# Autodesk Inventor assembly: ASY MSC 900.4  base frame
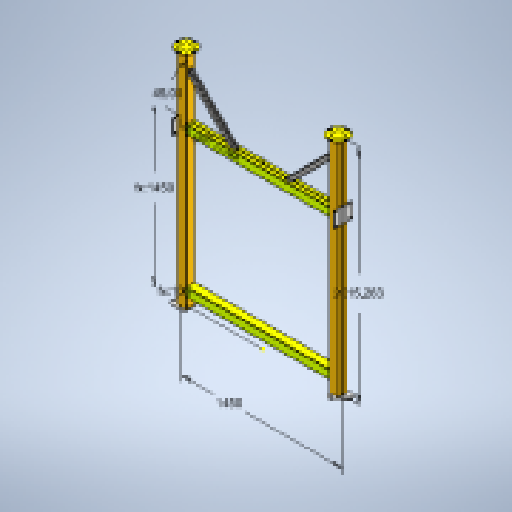
[picture p0: Inventor's stored thumbnail of the model, 512x512]
Saved by Autodesk Inventor 2025 (Build 290162010, 162A)
## iProperties
Created: 2024-06-30
Part Number: ASY MSC 900.4  base frame
Document SubType Name: Assembly
Designer: pokla
Stock Number: ASY МОО 900.4 базовая рама
_SolveAssemblyDoc: Frame Generator Solve Assembly
_Version: 25.0.0
Author: pokla
## Documents named in this file (7)
- C:\Users\pokla\Documents\Inventor\Отстойник осветлитель\Manturovo_Se-clar-Gleb\Pillars\ASY MSC 900.4  base frame.iam
- C:\Users\pokla\Documents\Inventor\Отстойник осветлитель\Manturovo_Se-clar-Gleb\Pillars\MSC DIM 009.4 base frame sketch.ipt
- C:\Users\pokla\Documents\Inventor\Отстойник осветлитель\Manturovo_Se-clar-Gleb\MSC 902 flange frame heel.ipt
- C:\Users\pokla\Documents\Inventor\Отстойник осветлитель\Manturovo_Se-clar-Gleb\MSC 906 flange frame.ipt
- C:\Users\pokla\Documents\Inventor\Отстойник осветлитель\Manturovo_Se-clar-Gleb\Pillars\Frame 1725454009874.iam
- C:\Users\pokla\Documents\Inventor\Отстойник осветлитель\Manturovo_Se-clar-Gleb\MSC DIM 000 settler-clarifier.ipt
- C:\Users\pokla\Documents\Inventor\Отстойник осветлитель\Manturovo_Se-clar-Gleb\MSC 908 transverse pillar plate.ipt
## Components (9 placed, 6 different names)
1. MSC DIM 009.4 base frame sketch:1
2. MSC 902 flange frame heel:1 — Rigid:2
3. MSC 902 flange frame heel:2 — Rigid:3
4. MSC 906 flange frame:1 — Rigid:4
5. MSC 906 flange frame:2 — Rigid:1
6. Frame 1725454009874:1 [sub-assembly] — Rigid:1, Rigid:2, Rigid:3, Rigid:4, Rigid:5, Rigid:6
7. MSC DIM 000 settler-clarifier:1
8. MSC 908 transverse pillar plate:1 — Rigid:5
9. MSC 908 transverse pillar plate:2 — Rigid:6
## Relationships (6: WeldJoint 6)
- Rigid:1 [WeldJoint]: MSC 906 flange frame:2 ↔ Frame 1725454009874:1
- Rigid:2 [WeldJoint]: MSC 902 flange frame heel:1 ↔ Frame 1725454009874:1
- Rigid:3 [WeldJoint]: MSC 902 flange frame heel:2 ↔ Frame 1725454009874:1
- Rigid:4 [WeldJoint]: MSC 906 flange frame:1 ↔ Frame 1725454009874:1
- Rigid:5 [WeldJoint] (80 mm): Frame 1725454009874:1 ↔ MSC 908 transverse pillar plate:1
- Rigid:6 [WeldJoint] (80 mm): Frame 1725454009874:1 ↔ MSC 908 transverse pillar plate:2
